# Autodesk Inventor assembly: assemble
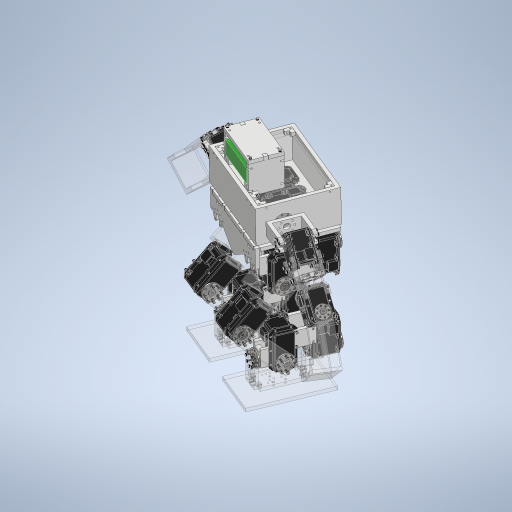
[picture p0: Inventor's stored thumbnail of the model, 512x512]
Saved by Autodesk Inventor 2024 (Build 280153000, 153)
## iProperties
Created: 2024-09-18
Part Number: assemble
Document SubType Name: Assembly
Designer: Eungang
Author: Eungang
## Documents named in this file (9)
- C:\Users\Eungang\Documents\Inventor\FIGHTING_ROBOT_FINAL\assemble.iam
- C:\Users\Eungang\Documents\Inventor\FIGHTING_ROBOT_FINAL\부품\Arm_Right\Right_Arm.iam
- C:\Users\Eungang\Documents\Inventor\FIGHTING_ROBOT_FINAL\부품\Upper_Leg_Left\Upper_Leg_Left.iam
- C:\Users\Eungang\Documents\Inventor\FIGHTING_ROBOT_FINAL\부품\Upper_Leg_Right\Upper_Leg_Right.iam
- C:\Users\Eungang\Documents\Inventor\FIGHTING_ROBOT_FINAL\부품\Waist-Chest\Waist.iam
- C:\Users\Eungang\Documents\Inventor\FIGHTING_ROBOT_FINAL\부품\Lower_Leg_Left\Lower_Leg_Left.iam
- C:\Users\Eungang\Documents\Inventor\FIGHTING_ROBOT_FINAL\부품\Arm_Left\Arm_Left.iam
- C:\Users\Eungang\Documents\Inventor\FIGHTING_ROBOT_FINAL\부품\Lower_Leg_Right\Lower_Leg_Right.iam
- C:\Users\Eungang\Documents\Inventor\FIGHTING_ROBOT_FINAL\부품\Head\Head.iam
## Components (8 placed, 8 different names)
1. Arm_Left:1 [sub-assembly] — 삽입:6
2. Right_Arm:1 [sub-assembly] — 삽입:5
3. Waist:1 [sub-assembly] — 삽입:3, 삽입:4, 삽입:5, 삽입:6, 삽입:7, 삽입:8
4. Upper_Leg_Left:1 [sub-assembly] — 삽입:1, 삽입:3
5. Lower_Leg_Left:1 [sub-assembly] — 메이트:1, 메이트:3, 삽입:2
6. Lower_Leg_Right:1 [sub-assembly] — 메이트:2, 메이트:3, 삽입:1
7. Upper_Leg_Right:1 [sub-assembly] — 삽입:2, 삽입:4
8. Head:1 [sub-assembly] — 삽입:7, 삽입:8
## Relationships (11: Insert 8, Mate 3)
- 메이트:1 [Mate]: Lower_Leg_Left:1
- 메이트:2 [Mate]: Lower_Leg_Right:1
- 메이트:3 [Mate]: Lower_Leg_Left:1 ↔ Lower_Leg_Right:1
- 삽입:1 [Insert] (0.1 mm): Upper_Leg_Left:1 ↔ Lower_Leg_Right:1
- 삽입:2 [Insert] (0.1 mm): Lower_Leg_Left:1 ↔ Upper_Leg_Right:1
- 삽입:3 [Insert]: Waist:1 ↔ Upper_Leg_Left:1
- 삽입:4 [Insert]: Waist:1 ↔ Upper_Leg_Right:1
- 삽입:5 [Insert]: Right_Arm:1 ↔ Waist:1
- 삽입:6 [Insert]: Arm_Left:1 ↔ Waist:1
- 삽입:7 [Insert] (0.2 mm): Waist:1 ↔ Head:1
- 삽입:8 [Insert] (0.2 mm): Waist:1 ↔ Head:1
